# Autodesk Inventor assembly: FlexK7V2
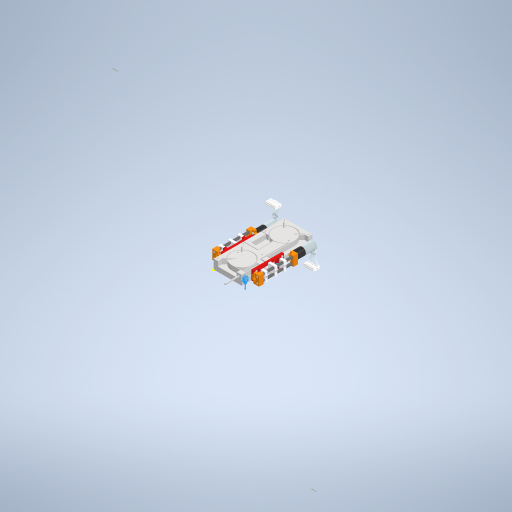
[picture p0: Inventor's stored thumbnail of the model, 512x512]
Saved by Autodesk Inventor 2023 (Build 270158000, 158)
## iProperties
Created: 2023-03-29
Part Number: FlexK7V2
Document SubType Name: Assembly
Designer: Nathann
Author: Nathann
## Documents named in this file (5)
- C:\Users\Nathann\ClawdDrive\Objet3D\IminaProbe\V2\FlexK7V2.iam
- C:\Users\Nathann\ClawdDrive\Objet3D\IminaProbe\V2\DifferentialLinearActuator.ipt
- C:\Users\Nathann\ClawdDrive\Objet3D\IminaProbe\V2\FlexK7V2.ipt
- C:\Users\Nathann\ClawdDrive\Objet3D\IminaProbe\V2\FlexK7Holder.ipt
- C:\Users\Nathann\ClawdDrive\Objet3D\3DPrinter\inventor\CapacitiveSensor.ipt
## Components (5 placed, 4 different names)
1. DifferentialLinearActuator:1 — Mate:1, Flush:1, Flush:2
2. DifferentialLinearActuator:2 — Mate:2, Flush:3, Flush:4
3. FlexK7V2:1 — Mate:1, Flush:1, Flush:2, Mate:2, Flush:3, Flush:4, Flush:5, Mate:3, Flush:6
4. FlexK7Holder:1 — Flush:5, Mate:3, Flush:6, Flush:7, Mate:4
5. CapacitiveSensor:1
## Relationships (11: Flush 7, Mate 4)
- Mate:1: DifferentialLinearActuator:1 ↔ FlexK7V2:1
- Flush:1 (-20 mm): DifferentialLinearActuator:1 ↔ FlexK7V2:1
- Flush:2: DifferentialLinearActuator:1 ↔ FlexK7V2:1
- Mate:2: DifferentialLinearActuator:2 ↔ FlexK7V2:1
- Flush:3: DifferentialLinearActuator:2 ↔ FlexK7V2:1
- Flush:4 (20 mm): DifferentialLinearActuator:2 ↔ FlexK7V2:1
- Flush:5: FlexK7V2:1 ↔ FlexK7Holder:1
- Mate:3: FlexK7V2:1 ↔ FlexK7Holder:1
- Flush:6: FlexK7V2:1 ↔ FlexK7Holder:1
- Flush:7: FlexK7Holder:1
- Mate:4: FlexK7Holder:1
